# Autodesk Inventor assembly: Potenciometro10K
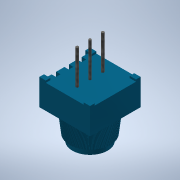
[picture p0: Inventor's stored thumbnail of the model, 180x180]
Saved by Autodesk Inventor 2022 (Build 260153000, 153)
## iProperties
Created: 2013-06-26
Part Number: Potenciometro10K
Document SubType Name: Assembly
Designer: usuario
Author: usuario
## Documents named in this file (3)
- C:\Users\JK\Documents\Inventor\N20 Leg Actuator\CADfiles\Potenciometro10K.iam
- C:\Users\JK\Documents\Inventor\N20 Leg Actuator\CADfiles\BasePotenciometro.ipt
- C:\Users\JK\Documents\Inventor\N20 Leg Actuator\CADfiles\PerillaPotenciometro.ipt
## Components (2 placed, 2 different names)
1. BasePotenciometro:1 — Insertar:1
2. PerillaPotenciometro:1 — Insertar:1
## Relationships (1: Insert 1)
- Insertar:1 (-1.98 mm): BasePotenciometro:1 ↔ PerillaPotenciometro:1
